# Autodesk Inventor assembly: pot1_assy
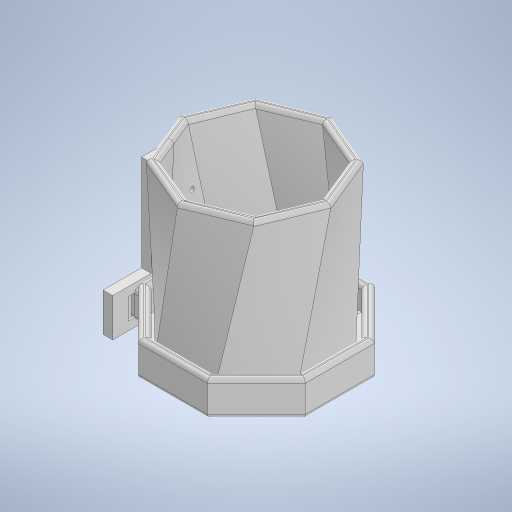
[picture p0: Inventor's stored thumbnail of the model, 512x512]
Saved by Autodesk Inventor 2023 (Build 270158000, 158)
## iProperties
Created: 2025-10-09
Part Number: pot1_assy
Document SubType Name: Assembly
Designer: Justin Pascual
Author: Justin Pascual
## Documents named in this file (5)
- C:\Users\Justin Pascual\Documents\GitHub\modular-flower-pot\pot1_assy.iam
- C:\Users\Justin Pascual\Documents\GitHub\modular-flower-pot\pot1.ipt
- C:\Users\Justin Pascual\Documents\GitHub\modular-flower-pot\dovetail.ipt
- C:\Users\Justin Pascual\Documents\GitHub\modular-flower-pot\base1.ipt
- C:\Users\Justin Pascual\Documents\GitHub\modular-flower-pot\mount1.ipt
## Components (5 placed, 4 different names)
1. pot1:1 — Mate:7, Mate:8, Flush:11, Mate:10, Mate:11
2. dovetail:1 — Mate:7, Mate:8, Mate:11, Mate:19, Mate:20, Mate:21
3. base1:1 — Flush:11, Mate:10, Mate:12, Mate:13, Mate:14
4. dovetail:2 — Mate:12, Mate:13, Mate:14, Mate:16, Mate:17, Mate:18
5. mount1:1 — Angle:1, Mate:15, Mate:16, Mate:17, Mate:18, Mate:19, Mate:20, Mate:21
## Relationships (16: Mate 14, Flush 1, Angle 1)
- Mate:7: pot1:1 ↔ dovetail:1
- Mate:8: pot1:1 ↔ dovetail:1
- Flush:11 (16.51 mm): pot1:1 ↔ base1:1
- Mate:10 (16.51 mm): pot1:1 ↔ base1:1
- Mate:11: pot1:1 ↔ dovetail:1
- Mate:12: base1:1 ↔ dovetail:2
- Mate:13: base1:1 ↔ dovetail:2
- Mate:14: base1:1 ↔ dovetail:2
- Angle:1 (180 deg): mount1:1
- Mate:15: mount1:1
- Mate:16 (0.508 mm): dovetail:2 ↔ mount1:1
- Mate:17: dovetail:2 ↔ mount1:1
- Mate:18 (3.81 mm): dovetail:2 ↔ mount1:1
- Mate:19: dovetail:1 ↔ mount1:1
- Mate:20: dovetail:1 ↔ mount1:1
- Mate:21: dovetail:1 ↔ mount1:1
